# Autodesk Inventor assembly: ASY GBK короткая стенка
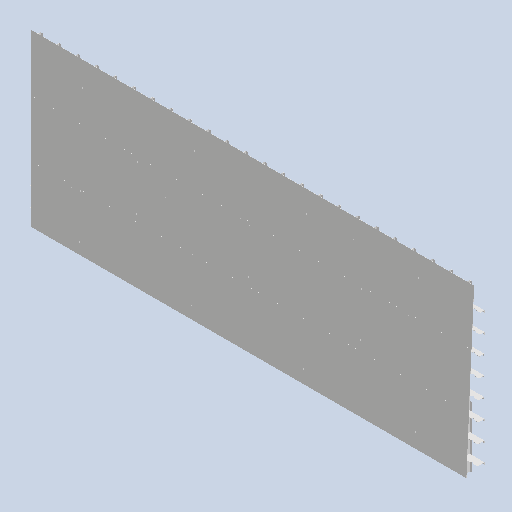
[picture p0: Inventor's stored thumbnail of the model, 512x512]
Saved by Autodesk Inventor 2026 (Build 300175000, 175)
## iProperties
Created: 2026-05-24
Part Number: ASY GBK короткая стенка
Document SubType Name: Assembly
Designer: pokla
Mass: 2.92121e+06 g
Surface Area: 1.88753e+06 cm^2
Volume: 372128 cm^3
Density: 7.85 g/cm^3
Author: pokla
## Documents named in this file (10)
- C:\Users\user\Documents\Inventor\GBK-Gubkinskiy\ASY GBK короткая стенка.iam
- C:\Users\user\Documents\Inventor\GBK-Gubkinskiy\ASY GBK 2110 short wall shield 1.iam
- C:\Users\user\Documents\Inventor\GBK-Gubkinskiy\ASY GBK 2120 short wall shield 2.iam
- C:\Users\user\Documents\Inventor\GBK-Gubkinskiy\ASY GBK 2130 short wall shield 3.iam
- C:\Users\user\Documents\Inventor\GBK-Gubkinskiy\ASY GBK 2210 short wall shield 4.iam
- C:\Users\user\Documents\Inventor\GBK-Gubkinskiy\ASY GBK 2310 short wall shield 7.iam
- C:\Users\user\Documents\Inventor\GBK-Gubkinskiy\ASY GBK 2320 short wall shield 8.iam
- C:\Users\user\Documents\Inventor\GBK-Gubkinskiy\ASY GBK 2330 short wall shield 9.iam
- C:\Users\user\Documents\Inventor\GBK-Gubkinskiy\ASY GBK 2220 short wall shield 5.iam
- C:\Users\user\Documents\Inventor\GBK-Gubkinskiy\ASY GBK 2230 short wall shield 6.iam
## Components (14 placed, 9 different names)
1. ASY GBK 2110 short wall shield 1.iam:1 [sub-assembly] — Жесткий:1, Заподлицо:1, Заподлицо:2, Совмещение:1
2. ASY GBK 2120 short wall shield 2.iam:1 [sub-assembly] — Жесткий:1, Жесткий:2
3. ASY GBK 2120 short wall shield 2.iam:2 [sub-assembly] — Жесткий:2, Жесткий:3
4. ASY GBK 2120 short wall shield 2.iam:3 [sub-assembly] — Жесткий:3, Жесткий:14
5. ASY GBK 2130 short wall shield 3.iam:1 [sub-assembly] — Жесткий:14, Заподлицо:3, Совмещение:2, Совмещение:4
6. ASY GBK 2210 short wall shield 4.iam:1 [sub-assembly] — Жесткий:17
7. ASY GBK 2220 short wall shield 5.iam:1 [sub-assembly] — Жесткий:7, Жесткий:17
8. ASY GBK 2220 short wall shield 5.iam:2 [sub-assembly] — Жесткий:7, Жесткий:16
9. ASY GBK 2230 short wall shield 6.iam:1 [sub-assembly] — Заподлицо:3, Совмещение:2, Заподлицо:5, Совмещение:3, Совмещение:4, Совмещение:5, Жесткий:16
10. ASY GBK 2310 short wall shield 7.iam:1 [sub-assembly] — Жесткий:10
11. ASY GBK 2320 short wall shield 8.iam:1 [sub-assembly] — Жесткий:10, Жесткий:11
12. ASY GBK 2330 short wall shield 9.iam:1 [sub-assembly] — Заподлицо:5, Совмещение:3, Совмещение:5, Жесткий:15
13. ASY GBK 2320 short wall shield 8.iam:2 [sub-assembly] — Жесткий:11, Жесткий:12
14. ASY GBK 2320 short wall shield 8.iam:3 [sub-assembly] — Жесткий:12, Жесткий:15
## Relationships (20: WeldJoint 11, Mate 5, Flush 4)
- Жесткий:1 [WeldJoint] (1 mm): ASY GBK 2110 short wall shield 1.iam:1 ↔ ASY GBK 2120 short wall shield 2.iam:1
- Жесткий:2 [WeldJoint] (1 mm): ASY GBK 2120 short wall shield 2.iam:1 ↔ ASY GBK 2120 short wall shield 2.iam:2
- Жесткий:3 [WeldJoint] (1 mm): ASY GBK 2120 short wall shield 2.iam:2 ↔ ASY GBK 2120 short wall shield 2.iam:3
- Жесткий:7 [WeldJoint] (1 mm): ASY GBK 2220 short wall shield 5.iam:1 ↔ ASY GBK 2220 short wall shield 5.iam:2
- Жесткий:10 [WeldJoint] (1 mm): ASY GBK 2310 short wall shield 7.iam:1 ↔ ASY GBK 2320 short wall shield 8.iam:1
- Жесткий:11 [WeldJoint] (1 mm): ASY GBK 2320 short wall shield 8.iam:1 ↔ ASY GBK 2320 short wall shield 8.iam:2
- Жесткий:12 [WeldJoint] (1 mm): ASY GBK 2320 short wall shield 8.iam:2 ↔ ASY GBK 2320 short wall shield 8.iam:3
- Заподлицо:1 [Flush]: ASY GBK 2110 short wall shield 1.iam:1
- Заподлицо:2 [Flush]: ASY GBK 2110 short wall shield 1.iam:1
- Совмещение:1 [Mate]: ASY GBK 2110 short wall shield 1.iam:1
- Жесткий:14 [WeldJoint] (1 mm): ASY GBK 2120 short wall shield 2.iam:3 ↔ ASY GBK 2130 short wall shield 3.iam:1
- Заподлицо:3 [Flush]: ASY GBK 2130 short wall shield 3.iam:1 ↔ ASY GBK 2230 short wall shield 6.iam:1
- Совмещение:2 [Mate] (1 mm): ASY GBK 2130 short wall shield 3.iam:1 ↔ ASY GBK 2230 short wall shield 6.iam:1
- Заподлицо:5 [Flush]: ASY GBK 2230 short wall shield 6.iam:1 ↔ ASY GBK 2330 short wall shield 9.iam:1
- Совмещение:3 [Mate] (1 mm): ASY GBK 2230 short wall shield 6.iam:1 ↔ ASY GBK 2330 short wall shield 9.iam:1
- Совмещение:4 [Mate] (1 mm): ASY GBK 2130 short wall shield 3.iam:1 ↔ ASY GBK 2230 short wall shield 6.iam:1
- Совмещение:5 [Mate] (1 mm): ASY GBK 2230 short wall shield 6.iam:1 ↔ ASY GBK 2330 short wall shield 9.iam:1
- Жесткий:15 [WeldJoint] (1 mm): ASY GBK 2330 short wall shield 9.iam:1 ↔ ASY GBK 2320 short wall shield 8.iam:3
- Жесткий:16 [WeldJoint] (1 mm): ASY GBK 2220 short wall shield 5.iam:2 ↔ ASY GBK 2230 short wall shield 6.iam:1
- Жесткий:17 [WeldJoint] (1 mm): ASY GBK 2210 short wall shield 4.iam:1 ↔ ASY GBK 2220 short wall shield 5.iam:1
